# Autodesk Inventor assembly: IG28-014-035
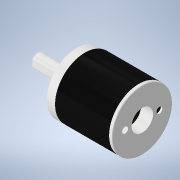
[picture p0: Inventor's stored thumbnail of the model, 180x180]
Saved by Autodesk Inventor 2022 (Build 260153000, 153)
## iProperties
Created: 2018-06-27
Part Number: IG28-014-035
Document SubType Name: Assembly
Designer: YusukeKunita
Mass: 81 g
Surface Area: 98.0874 cm^2
Volume: 9.19325 cm^3
Title: /vol/tmp/translate-6351052721594182796/5b330ce725b7221395fdb4df.step
Revision Number: NONE
## Documents named in this file (5)
- C:\Users\YusukeKunita\Documents\GrabCAD\NHK2022\BasicParts\Motor\GearHead\IG28-014-035\IG28-014-035.iam
- C:\Users\YusukeKunita\Documents\GrabCAD\NHK2022\BasicParts\Motor\GearHead\IG28-014-035\Part 1.ipt
- C:\Users\YusukeKunita\Documents\GrabCAD\NHK2022\BasicParts\Motor\GearHead\IG28-014-035\Part 1_1.ipt
- C:\Users\YusukeKunita\Documents\GrabCAD\NHK2022\BasicParts\Motor\GearHead\IG28-014-035\Part 1_2.ipt
- C:\Users\YusukeKunita\Documents\GrabCAD\NHK2022\BasicParts\Motor\GearHead\IG28-014-035\Part 1_3.ipt
## Components (4 placed, 4 different names)
1. NAUO1 — 回転:1
2. NAUO2 — 回転:3
3. NAUO3 — 回転:2, 回転:3
4. NAUO4 — 回転:1, 回転:2
## Relationships (3: RevoluteJoint 3)
- 回転:1 [RevoluteJoint]: NAUO1 ↔ NAUO4
- 回転:2 [RevoluteJoint]: NAUO3 ↔ NAUO4
- 回転:3 [RevoluteJoint] (18.1 mm): NAUO2 ↔ NAUO3
